# Autodesk Inventor assembly: springPusherAssembly
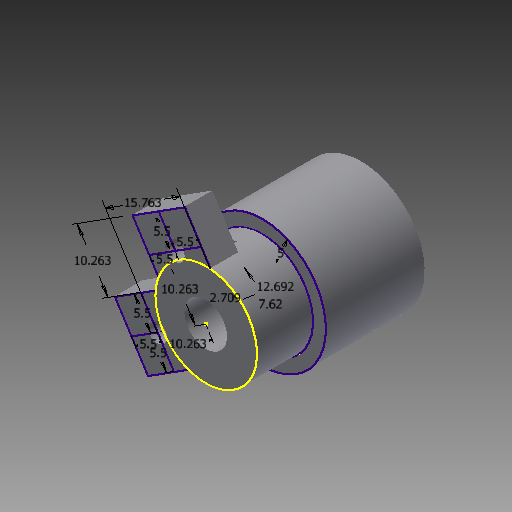
[picture p0: Inventor's stored thumbnail of the model, 512x512]
Saved by Autodesk Inventor 2018 (Build 220112000, 112)
## iProperties
Created: 2017-11-09
Part Number: springPusherAssembly
Document SubType Name: Assembly
Designer: Payal Jindal
Author: Payal Jindal
## Documents named in this file (3)
- C:\Users\Prakash\Documents\Inventor\MousetrapGit\springPusherAssembly.iam
- C:\Users\Prakash\Documents\Inventor\MousetrapGit\9001T180_MUSIC WIRE ULTRA-PRECISION COMPRESSION SPRING.ipt
- C:\Users\Prakash\Documents\Inventor\MousetrapGit\springHolder_final.ipt
## Components (2 placed, 2 different names)
1. 9001T180_MUSIC WIRE ULTRA-PRECISION COMPRESSION SPRING:1 — Mate:3, Mate:4, Mate:5
2. springHolder_final:1 — Mate:3, Mate:4, Mate:5
## Relationships (3: Mate 3)
- Mate:3: 9001T180_MUSIC WIRE ULTRA-PRECISION COMPRESSION SPRING:1 ↔ springHolder_final:1
- Mate:4: 9001T180_MUSIC WIRE ULTRA-PRECISION COMPRESSION SPRING:1 ↔ springHolder_final:1
- Mate:5: 9001T180_MUSIC WIRE ULTRA-PRECISION COMPRESSION SPRING:1 ↔ springHolder_final:1
